# Autodesk Inventor assembly: Assembly1
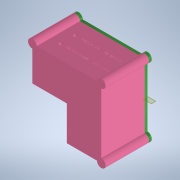
[picture p0: Inventor's stored thumbnail of the model, 180x180]
Saved by Autodesk Inventor 2020 (Build 240168000, 168)
## iProperties
Created: 2019-12-06
Part Number: Assembly1
Document SubType Name: Assembly
Designer: Alex
Author: Alex
## Documents named in this file (4)
- C:\Users\Alex\Documents\Inventor\PLD_ALarm\Assembly1.iam
- C:\Users\Alex\Documents\Inventor\PLD_ALarm\Deckel.ipt
- C:\Users\Alex\Documents\Inventor\PLD_ALarm\Ring_New.ipt
- C:\Users\Alex\Documents\Inventor\PLD_ALarm\Case.ipt
## Components (3 placed, 3 different names)
1. Case:1 — Rotational:3, Rotational:4
2. Deckel:1 — Rotational:1, Rotational:2, Rotational:3, Rotational:4
3. Ring_New:1 — Rotational:1, Rotational:2
## Relationships (4: RevoluteJoint 4)
- Rotational:1 [RevoluteJoint]: Deckel:1 ↔ Ring_New:1
- Rotational:2 [RevoluteJoint]: Deckel:1 ↔ Ring_New:1
- Rotational:3 [RevoluteJoint]: Case:1 ↔ Deckel:1
- Rotational:4 [RevoluteJoint]: Case:1 ↔ Deckel:1
